# Autodesk Inventor assembly: Wrist
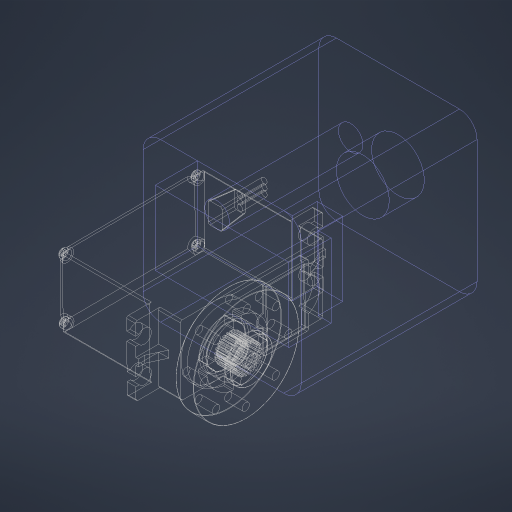
[picture p0: Inventor's stored thumbnail of the model, 512x512]
Saved by Autodesk Inventor 2023 (Build 270158000, 158)
## iProperties
Created: 2023-04-10
Part Number: Wrist
Document SubType Name: Assembly
Designer: vatdu
Author: vatdu
## Documents named in this file (4)
- C:\Users\vatdu\Desktop\CRYSTAL MARK II\Arm\Wrist\Wrist.iam
- C:\Users\vatdu\Desktop\CRYSTAL MARK II\Arm\Wrist\Motor holder.ipt
- C:\Users\vatdu\Desktop\CRYSTAL MARK II\Components\Servo.ipt
- C:\Users\vatdu\Desktop\CRYSTAL MARK II\Components\Arm_Disc.ipt
## Components (3 placed, 3 different names)
1. Motor holder:1
2. Servo:1 — Rotational:1
3. Arm_Disc:1 — Rotational:1
## Relationships (1: RevoluteJoint 1)
- Rotational:1 [RevoluteJoint] (3.5 mm): Servo:1 ↔ Arm_Disc:1
